# Autodesk Inventor assembly: SPE1V1 Estructura
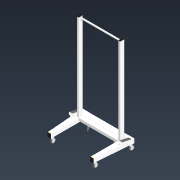
[picture p0: Inventor's stored thumbnail of the model, 180x180]
Saved by Autodesk Inventor 2021.2 (Build 252289000, 289)
## iProperties
Created: 2026-06-02
Part Number: SPE1V1 Estructura
Document SubType Name: Assembly
Designer: nelso
Mass: 32774.5 g
Surface Area: 45303.3 cm^2
Volume: 6303.93 cm^3
Density: 5.19906 g/cm^3
Author: nelso
## Documents named in this file (22)
- C:\Users\Tecnica\OneDrive\Documentos\Mecanica\Soporte-Paciente-Espinografia\Workspace\SPE1V1 Estructura.iam
- C:\Users\Tecnica\OneDrive\Documentos\Mecanica\Soporte-Paciente-Espinografia\Workspace\SP19V1 Tapacanto Delantero.ipt
- C:\Users\Tecnica\OneDrive\Documentos\Mecanica\Soporte-Paciente-Espinografia\Workspace\SP18V1 Tapacanto Superior.ipt
- C:\Users\Tecnica\OneDrive\Documentos\Mecanica\Soporte-Paciente-Espinografia\Workspace\RFPLUS8PO300.ipt
- C:\Users\Tecnica\OneDrive\Documentos\Mecanica\Soporte-Paciente-Espinografia\Workspace\SP17V1 Varilla Pedal.ipt
- C:\Users\Tecnica\OneDrive\Documentos\Mecanica\Soporte-Paciente-Espinografia\Workspace\SP15V1 Pedal Izquierdo.ipt
- C:\Users\Tecnica\OneDrive\Documentos\Mecanica\Soporte-Paciente-Espinografia\Workspace\SPE3V1 Freno.iam
- C:\Users\Tecnica\OneDrive\Documentos\Mecanica\Soporte-Paciente-Espinografia\Workspace\SP14V1 Pedal Derecho.ipt
- C:\Users\Tecnica\OneDrive\Documentos\Mecanica\Soporte-Paciente-Espinografia\Workspace\G3-100-PPP-RU.ipt
- C:\Users\Tecnica\OneDrive\Documentos\Mecanica\Soporte-Paciente-Espinografia\Workspace\DIN 555A10C.ipt
- C:\Users\Tecnica\OneDrive\Documentos\Mecanica\Soporte-Paciente-Espinografia\Workspace\DIN125-A8,4C.ipt
- C:\Users\Tecnica\OneDrive\Documentos\Mecanica\Soporte-Paciente-Espinografia\Workspace\DIN933M8X1.25L20C.ipt
- C:\Users\Tecnica\OneDrive\Documentos\Mecanica\Soporte-Paciente-Espinografia\Workspace\SP11V1 Planchuela Baranda.ipt
- C:\Users\Tecnica\OneDrive\Documentos\Mecanica\Soporte-Paciente-Espinografia\Workspace\SP52V1 Tubo superior.ipt
- C:\Users\Tecnica\OneDrive\Documentos\Mecanica\Soporte-Paciente-Espinografia\Workspace\SP58V1 Seguro Pedales.ipt
- C:\Users\Tecnica\OneDrive\Documentos\Mecanica\Soporte-Paciente-Espinografia\Workspace\ISO7380M6X1L12I.ipt
- C:\Users\Tecnica\OneDrive\Documentos\Mecanica\Soporte-Paciente-Espinografia\Workspace\DIN137-B6.ipt
- C:\Users\Tecnica\OneDrive\Documentos\Mecanica\Soporte-Paciente-Espinografia\Workspace\ISO7380M4X0.8L12I.ipt
- C:\Users\Tecnica\OneDrive\Documentos\Mecanica\Soporte-Paciente-Espinografia\Workspace\DIN137-B4.ipt
- C:\Users\Tecnica\OneDrive\Documentos\Mecanica\Soporte-Paciente-Espinografia\Workspace\DIN555-5M4X0.8I.ipt
- C:\Users\Tecnica\OneDrive\Documentos\Mecanica\Soporte-Paciente-Espinografia\Workspace\SP59V1 Goma Pedalesl.ipt
- C:\Users\Tecnica\OneDrive\Documentos\Mecanica\Soporte-Paciente-Espinografia\Workspace\SPE61V1 Estructura (soldadura).iam
## Components (69 placed, 21 different names)
1. SP18V1 Tapacanto Superior:1
2. SP18V1 Tapacanto Superior:2
3. SP19V1 Tapacanto Delantero:1
4. SP19V1 Tapacanto Delantero:2
5. RFPLUS8PO300:1
6. RFPLUS8PO300:2
7. RFPLUS8PO300:3
8. RFPLUS8PO300:4
9. RFPLUS8PO300:5
10. RFPLUS8PO300:6
11. SP17V1 Varilla Pedal:1 — Mate:117, Mate:118, Mate:119, Mate:120, Mate:121, Mate:128, Mate:129, Mate:130, Mate:132, Mate:133, Mate:134, Mate:258, Mate:261
12. SP14V1 Pedal Derecho:1 — Mate:128, Mate:129, Mate:130, Mate:132, Mate:200, Mate:251, Mate:252, Mate:253, Mate:292, Mate:293, Mate:294, Mate:295, Mate:296
13. SP15V1 Pedal Izquierdo:1 — Mate:120, Mate:121, Flush:132, Mate:248, Mate:249, Mate:250, Mate:286, Mate:287, Mate:297, Mate:298, Mate:299
14. SPE3V1 Freno:1 [sub-assembly] — Flush:103, Mate:117, Mate:118, Mate:119
15. SPE3V1 Freno:2 [sub-assembly] — Flush:103, Mate:133, Mate:134
16. RFPLUS8PO300:17
17. RFPLUS8PO300:18
18. RFPLUS8PO300:19
19. RFPLUS8PO300:20
20. RFPLUS8PO300:21
21. RFPLUS8PO300:22
22. G3-100-PPP-RU:1
23. G3-100-PPP-RU:2
24. G3-100-PPP-RU:3
25. G3-100-PPP-RU:4
26. DIN 555A10C:1
27. DIN 555A10C:2
28. DIN 555A10C:3
29. DIN 555A10C:4
30. DIN125-A8,4C:1 — Mate:214, Mate:215, Mate:219
31. DIN933M8X1.25L20C:1 — Mate:214, Mate:215, Mate:220, Mate:224
32. SP11V1 Planchuela Baranda:1 — Mate:218, Mate:219, Mate:220, Mate:221
33. DIN125-A8,4C:2 — Mate:216, Mate:217, Mate:218
34. DIN933M8X1.25L20C:2 — Mate:216, Mate:217, Mate:221, Mate:223
35. RFPLUS8PO300:23 — Mate:223
36. RFPLUS8PO300:24 — Mate:224
37. DIN125-A8,4C:3
38. DIN933M8X1.25L20C:3
39. SP11V1 Planchuela Baranda:2 — Mate:241
40. DIN125-A8,4C:4
41. DIN933M8X1.25L20C:4
42. RFPLUS8PO300:25
43. RFPLUS8PO300:26
44. SP52V1 Tubo superior:1 — Mate:240, Mate:241
45. SP58V1 Seguro Pedales:1 — Mate:248, Mate:249, Mate:250, Mate:260, Mate:274, Mate:275, Mate:276, Mate:277
46. SP58V1 Seguro Pedales:2 — Mate:251, Mate:252, Mate:253, Mate:259, Mate:270, Mate:271, Mate:272, Mate:273
47. ISO7380M6X1L12I:1 — Mate:254, Mate:255, Mate:258
48. DIN137-B6:1 — Mate:254, Mate:255, Mate:259
49. ISO7380M6X1L12I:2 — Mate:261
50. DIN137-B6:2 — Mate:260
51. ISO7380M4X0.8L12I:1 — Mate:264, Mate:265, Mate:277, Mate:278, Mate:282
52. ISO7380M4X0.8L12I:2 — Mate:262, Mate:263, Mate:276, Mate:279, Mate:284
53. ISO7380M4X0.8L12I:3 — Mate:266, Mate:267, Mate:273, Mate:281, Mate:288
54. ISO7380M4X0.8L12I:4 — Mate:268, Mate:269, Mate:272, Mate:280, Mate:289
55. DIN137-B4:1 — Mate:262, Mate:263, Mate:275
56. DIN137-B4:2 — Mate:264, Mate:265, Mate:274
57. DIN137-B4:3 — Mate:268, Mate:269, Mate:270
58. DIN137-B4:4 — Mate:266, Mate:267, Mate:271
59. DIN137-B4:5 — Mate:279, Mate:285, Mate:287
60. DIN137-B4:6 — Mate:278, Mate:283, Mate:286
61. DIN137-B4:7 — Mate:280, Mate:290, Mate:293
62. DIN137-B4:8 — Mate:281, Mate:291, Mate:292
63. DIN555-5M4X0.8I:1 — Mate:282, Mate:283
64. DIN555-5M4X0.8I:2 — Mate:284, Mate:285
65. DIN555-5M4X0.8I:3 — Mate:289, Mate:290
66. DIN555-5M4X0.8I:4 — Mate:288, Mate:291
67. SP59V1 Goma Pedalesl:1 — Mate:294, Mate:295, Mate:296
68. SP59V1 Goma Pedalesl:2 — Mate:297, Mate:298, Mate:299
69. SPE61V1 Estructura (soldadura):1 [sub-assembly]
## Relationships (168: Mate 134, Flush 33, Angle 1)
- [Mate]: SP18V1 Tapacanto Superior:1 ↔ SPE61V1 Estructura (soldadura):1
- [Flush]: SP18V1 Tapacanto Superior:1 ↔ SPE61V1 Estructura (soldadura):1
- [Mate]: SP18V1 Tapacanto Superior:1 ↔ SPE61V1 Estructura (soldadura):1
- [Flush]: RFPLUS8PO300:2 ↔ SPE61V1 Estructura (soldadura):1
- [Flush]: RFPLUS8PO300:3 ↔ SPE61V1 Estructura (soldadura):1
- [Flush]: RFPLUS8PO300:4 ↔ SPE61V1 Estructura (soldadura):1
- [Flush]: RFPLUS8PO300:5 ↔ SPE61V1 Estructura (soldadura):1
- [Flush]: RFPLUS8PO300:6 ↔ SPE61V1 Estructura (soldadura):1
- [Mate]: RFPLUS8PO300:5 ↔ SPE61V1 Estructura (soldadura):1
- [Mate]: RFPLUS8PO300:6 ↔ SPE61V1 Estructura (soldadura):1
- [Mate]: RFPLUS8PO300:4 ↔ SPE61V1 Estructura (soldadura):1
- [Mate]: RFPLUS8PO300:3 ↔ SPE61V1 Estructura (soldadura):1
- [Mate]: RFPLUS8PO300:2 ↔ SPE61V1 Estructura (soldadura):1
- [Mate]: RFPLUS8PO300:1 ↔ SPE61V1 Estructura (soldadura):1
- [Flush]: RFPLUS8PO300:1 ↔ SPE61V1 Estructura (soldadura):1
- [Mate]: SPE3V1 Freno:1 ↔ SPE61V1 Estructura (soldadura):1
- [Mate]: SPE3V1 Freno:2 ↔ SPE61V1 Estructura (soldadura):1
- Flush:103: SPE3V1 Freno:1 ↔ SPE3V1 Freno:2
- Mate:117: SP17V1 Varilla Pedal:1 ↔ SPE3V1 Freno:1
- Mate:118: SP17V1 Varilla Pedal:1 ↔ SPE3V1 Freno:1
- Mate:119: SP17V1 Varilla Pedal:1 ↔ SPE3V1 Freno:1
- Mate:120: SP17V1 Varilla Pedal:1 ↔ SP15V1 Pedal Izquierdo:1
- Mate:121: SP17V1 Varilla Pedal:1 ↔ SP15V1 Pedal Izquierdo:1
- [Mate]: SPE3V1 Freno:1 ↔ SPE61V1 Estructura (soldadura):1
- [Mate]: SP17V1 Varilla Pedal:1 ↔ SPE61V1 Estructura (soldadura):1
- [Mate] (100 mm): SPE3V1 Freno:2 ↔ SPE61V1 Estructura (soldadura):1
- [Mate] (100 mm): SPE3V1 Freno:1 ↔ SPE61V1 Estructura (soldadura):1
- Mate:128: SP17V1 Varilla Pedal:1 ↔ SP14V1 Pedal Derecho:1
- Mate:129: SP17V1 Varilla Pedal:1 ↔ SP14V1 Pedal Derecho:1
- Mate:130: SP17V1 Varilla Pedal:1 ↔ SP14V1 Pedal Derecho:1
- Mate:132: SP17V1 Varilla Pedal:1 ↔ SP14V1 Pedal Derecho:1
- Mate:133: SP17V1 Varilla Pedal:1 ↔ SPE3V1 Freno:2
- Mate:134: SP17V1 Varilla Pedal:1 ↔ SPE3V1 Freno:2
- [Flush]: SP18V1 Tapacanto Superior:2 ↔ SPE61V1 Estructura (soldadura):1
- [Mate]: SP18V1 Tapacanto Superior:2 ↔ SPE61V1 Estructura (soldadura):1
- [Mate]: G3-100-PPP-RU:4 ↔ SPE61V1 Estructura (soldadura):1
- [Mate]: SP18V1 Tapacanto Superior:2 ↔ SPE61V1 Estructura (soldadura):1
- [Mate]: RFPLUS8PO300:21 ↔ SPE61V1 Estructura (soldadura):1
- [Mate]: RFPLUS8PO300:22 ↔ SPE61V1 Estructura (soldadura):1
- [Mate]: RFPLUS8PO300:20 ↔ SPE61V1 Estructura (soldadura):1
- [Mate]: RFPLUS8PO300:19 ↔ SPE61V1 Estructura (soldadura):1
- [Mate]: RFPLUS8PO300:18 ↔ SPE61V1 Estructura (soldadura):1
- [Mate]: RFPLUS8PO300:17 ↔ SPE61V1 Estructura (soldadura):1
- [Flush]: RFPLUS8PO300:17 ↔ SPE61V1 Estructura (soldadura):1
- [Flush]: RFPLUS8PO300:18 ↔ SPE61V1 Estructura (soldadura):1
- [Flush]: RFPLUS8PO300:19 ↔ SPE61V1 Estructura (soldadura):1
- [Flush]: RFPLUS8PO300:20 ↔ SPE61V1 Estructura (soldadura):1
- [Flush]: RFPLUS8PO300:21 ↔ SPE61V1 Estructura (soldadura):1
- [Flush]: RFPLUS8PO300:22 ↔ SPE61V1 Estructura (soldadura):1
- [Mate]: DIN 555A10C:3 ↔ SPE61V1 Estructura (soldadura):1
- [Mate]: DIN 555A10C:4 ↔ SPE61V1 Estructura (soldadura):1
- [Mate]: DIN 555A10C:2 ↔ SPE61V1 Estructura (soldadura):1
- [Mate]: DIN 555A10C:1 ↔ SPE61V1 Estructura (soldadura):1
- [Mate]: DIN 555A10C:1 ↔ SPE61V1 Estructura (soldadura):1
- [Mate]: DIN 555A10C:2 ↔ SPE61V1 Estructura (soldadura):1
- [Mate]: DIN 555A10C:3 ↔ SPE61V1 Estructura (soldadura):1
- [Mate]: DIN 555A10C:4 ↔ SPE61V1 Estructura (soldadura):1
- [Flush]: SP17V1 Varilla Pedal:1 ↔ SPE61V1 Estructura (soldadura):1
- [Flush] (7.5 mm): SPE61V1 Estructura (soldadura):1
- [Flush] (7.5 mm): SPE61V1 Estructura (soldadura):1
- Flush:132: SP15V1 Pedal Izquierdo:1
- Mate:200: SP14V1 Pedal Derecho:1
- [Mate]: G3-100-PPP-RU:3 ↔ SPE61V1 Estructura (soldadura):1
- [Mate]: G3-100-PPP-RU:3 ↔ SPE61V1 Estructura (soldadura):1
- [Flush]: G3-100-PPP-RU:3 ↔ SPE61V1 Estructura (soldadura):1
- [Mate]: G3-100-PPP-RU:2 ↔ SPE61V1 Estructura (soldadura):1
- [Mate]: G3-100-PPP-RU:2 ↔ SPE61V1 Estructura (soldadura):1
- [Flush]: G3-100-PPP-RU:2 ↔ SPE61V1 Estructura (soldadura):1
- [Mate]: G3-100-PPP-RU:4 ↔ SPE61V1 Estructura (soldadura):1
- [Flush]: G3-100-PPP-RU:4 ↔ SPE61V1 Estructura (soldadura):1
- [Mate]: G3-100-PPP-RU:1 ↔ SPE61V1 Estructura (soldadura):1
- [Flush]: G3-100-PPP-RU:1 ↔ SPE61V1 Estructura (soldadura):1
- [Mate]: G3-100-PPP-RU:1 ↔ SPE61V1 Estructura (soldadura):1
- [Mate]: SP19V1 Tapacanto Delantero:1 ↔ SPE61V1 Estructura (soldadura):1
- [Flush]: SPE61V1 Estructura (soldadura):1
- [Mate]: SPE61V1 Estructura (soldadura):1
- [Flush]: SPE61V1 Estructura (soldadura):1
- [Mate] (380 mm): SPE61V1 Estructura (soldadura):1
- [Flush]: SP19V1 Tapacanto Delantero:2 ↔ SPE61V1 Estructura (soldadura):1
- [Flush]: SP19V1 Tapacanto Delantero:2 ↔ SPE61V1 Estructura (soldadura):1
- [Mate]: SP19V1 Tapacanto Delantero:2 ↔ SPE61V1 Estructura (soldadura):1
- [Flush]: SP19V1 Tapacanto Delantero:1 ↔ SPE61V1 Estructura (soldadura):1
- [Flush]: SP19V1 Tapacanto Delantero:1 ↔ SPE61V1 Estructura (soldadura):1
- Mate:214: DIN125-A8,4C:1 ↔ DIN933M8X1.25L20C:1
- Mate:215: DIN125-A8,4C:1 ↔ DIN933M8X1.25L20C:1
- Mate:216: DIN125-A8,4C:2 ↔ DIN933M8X1.25L20C:2
- Mate:217: DIN125-A8,4C:2 ↔ DIN933M8X1.25L20C:2
- Mate:218: SP11V1 Planchuela Baranda:1 ↔ DIN125-A8,4C:2
- Mate:219: DIN125-A8,4C:1 ↔ SP11V1 Planchuela Baranda:1
- Mate:220: DIN933M8X1.25L20C:1 ↔ SP11V1 Planchuela Baranda:1
- Mate:221: SP11V1 Planchuela Baranda:1 ↔ DIN933M8X1.25L20C:2
- [Mate]: SP11V1 Planchuela Baranda:1 ↔ SPE61V1 Estructura (soldadura):1
- [Flush]: RFPLUS8PO300:24 ↔ SPE61V1 Estructura (soldadura):1
- [Flush]: RFPLUS8PO300:23 ↔ SPE61V1 Estructura (soldadura):1
- Mate:223: DIN933M8X1.25L20C:2 ↔ RFPLUS8PO300:23
- Mate:224: DIN933M8X1.25L20C:1 ↔ RFPLUS8PO300:24
- [Mate]: DIN125-A8,4C:3 ↔ DIN933M8X1.25L20C:3
- [Mate]: DIN125-A8,4C:3 ↔ DIN933M8X1.25L20C:3
- [Mate]: DIN125-A8,4C:4 ↔ DIN933M8X1.25L20C:4
- [Mate]: DIN125-A8,4C:4 ↔ DIN933M8X1.25L20C:4
- [Mate]: SP11V1 Planchuela Baranda:2 ↔ DIN125-A8,4C:4
- [Mate]: DIN125-A8,4C:3 ↔ SP11V1 Planchuela Baranda:2
- [Mate]: DIN933M8X1.25L20C:3 ↔ SP11V1 Planchuela Baranda:2
- [Mate]: SP11V1 Planchuela Baranda:2 ↔ DIN933M8X1.25L20C:4
- [Mate]: DIN933M8X1.25L20C:4 ↔ RFPLUS8PO300:25
- [Mate]: DIN933M8X1.25L20C:3 ↔ RFPLUS8PO300:26
- [Mate]: SP11V1 Planchuela Baranda:2 ↔ SPE61V1 Estructura (soldadura):1
- [Flush]: RFPLUS8PO300:26 ↔ SPE61V1 Estructura (soldadura):1
- [Flush]: RFPLUS8PO300:25 ↔ SPE61V1 Estructura (soldadura):1
- [Mate]: DIN933M8X1.25L20C:1 ↔ SPE61V1 Estructura (soldadura):1
- [Mate]: DIN933M8X1.25L20C:2 ↔ SPE61V1 Estructura (soldadura):1
- [Mate]: DIN933M8X1.25L20C:3 ↔ SPE61V1 Estructura (soldadura):1
- [Mate]: DIN933M8X1.25L20C:4 ↔ SPE61V1 Estructura (soldadura):1
- Mate:240: SP52V1 Tubo superior:1
- Mate:241: SP11V1 Planchuela Baranda:2 ↔ SP52V1 Tubo superior:1
- Mate:248: SP15V1 Pedal Izquierdo:1 ↔ SP58V1 Seguro Pedales:1
- Mate:249: SP15V1 Pedal Izquierdo:1 ↔ SP58V1 Seguro Pedales:1
- Mate:250: SP15V1 Pedal Izquierdo:1 ↔ SP58V1 Seguro Pedales:1
- Mate:251: SP14V1 Pedal Derecho:1 ↔ SP58V1 Seguro Pedales:2
- Mate:252: SP14V1 Pedal Derecho:1 ↔ SP58V1 Seguro Pedales:2
- Mate:253: SP14V1 Pedal Derecho:1 ↔ SP58V1 Seguro Pedales:2
- Mate:254: ISO7380M6X1L12I:1 ↔ DIN137-B6:1
- Mate:255: ISO7380M6X1L12I:1 ↔ DIN137-B6:1
- [Mate]: ISO7380M6X1L12I:2 ↔ DIN137-B6:2
- [Mate]: ISO7380M6X1L12I:2 ↔ DIN137-B6:2
- Mate:258: SP17V1 Varilla Pedal:1 ↔ ISO7380M6X1L12I:1
- Mate:259: SP58V1 Seguro Pedales:2 ↔ DIN137-B6:1
- Mate:260: SP58V1 Seguro Pedales:1 ↔ DIN137-B6:2
- Mate:261: SP17V1 Varilla Pedal:1 ↔ ISO7380M6X1L12I:2
- Mate:262: ISO7380M4X0.8L12I:2 ↔ DIN137-B4:1
- Mate:263: ISO7380M4X0.8L12I:2 ↔ DIN137-B4:1
- Mate:264: ISO7380M4X0.8L12I:1 ↔ DIN137-B4:2
- Mate:265: ISO7380M4X0.8L12I:1 ↔ DIN137-B4:2
- Mate:266: ISO7380M4X0.8L12I:3 ↔ DIN137-B4:4
- Mate:267: ISO7380M4X0.8L12I:3 ↔ DIN137-B4:4
- Mate:268: ISO7380M4X0.8L12I:4 ↔ DIN137-B4:3
- Mate:269: ISO7380M4X0.8L12I:4 ↔ DIN137-B4:3
- Mate:270: SP58V1 Seguro Pedales:2 ↔ DIN137-B4:3
- Mate:271: SP58V1 Seguro Pedales:2 ↔ DIN137-B4:4
- Mate:272: SP58V1 Seguro Pedales:2 ↔ ISO7380M4X0.8L12I:4
- Mate:273: SP58V1 Seguro Pedales:2 ↔ ISO7380M4X0.8L12I:3
- Mate:274: SP58V1 Seguro Pedales:1 ↔ DIN137-B4:2
- Mate:275: SP58V1 Seguro Pedales:1 ↔ DIN137-B4:1
- Mate:276: SP58V1 Seguro Pedales:1 ↔ ISO7380M4X0.8L12I:2
- Mate:277: SP58V1 Seguro Pedales:1 ↔ ISO7380M4X0.8L12I:1
- Mate:278: ISO7380M4X0.8L12I:1 ↔ DIN137-B4:6
- Mate:279: ISO7380M4X0.8L12I:2 ↔ DIN137-B4:5
- Mate:280: ISO7380M4X0.8L12I:4 ↔ DIN137-B4:7
- Mate:281: ISO7380M4X0.8L12I:3 ↔ DIN137-B4:8
- Mate:282: ISO7380M4X0.8L12I:1 ↔ DIN555-5M4X0.8I:1
- Mate:283: DIN137-B4:6 ↔ DIN555-5M4X0.8I:1
- Mate:284: ISO7380M4X0.8L12I:2 ↔ DIN555-5M4X0.8I:2
- Mate:285: DIN137-B4:5 ↔ DIN555-5M4X0.8I:2
- Mate:286: SP15V1 Pedal Izquierdo:1 ↔ DIN137-B4:6
- Mate:287: SP15V1 Pedal Izquierdo:1 ↔ DIN137-B4:5
- Mate:288: ISO7380M4X0.8L12I:3 ↔ DIN555-5M4X0.8I:4
- Mate:289: ISO7380M4X0.8L12I:4 ↔ DIN555-5M4X0.8I:3
- Mate:290: DIN137-B4:7 ↔ DIN555-5M4X0.8I:3
- Mate:291: DIN137-B4:8 ↔ DIN555-5M4X0.8I:4
- Mate:292: SP14V1 Pedal Derecho:1 ↔ DIN137-B4:8
- Mate:293: SP14V1 Pedal Derecho:1 ↔ DIN137-B4:7
- [Angle] (0 deg): SP14V1 Pedal Derecho:1 ↔ SPE61V1 Estructura (soldadura):1
- Mate:294: SP14V1 Pedal Derecho:1 ↔ SP59V1 Goma Pedalesl:1
- Mate:295: SP14V1 Pedal Derecho:1 ↔ SP59V1 Goma Pedalesl:1
- Mate:296: SP14V1 Pedal Derecho:1 ↔ SP59V1 Goma Pedalesl:1
- Mate:297: SP15V1 Pedal Izquierdo:1 ↔ SP59V1 Goma Pedalesl:2
- Mate:298: SP15V1 Pedal Izquierdo:1 ↔ SP59V1 Goma Pedalesl:2
- Mate:299: SP15V1 Pedal Izquierdo:1 ↔ SP59V1 Goma Pedalesl:2
## Named parameters: d314_d103 = 0 mm, d315_d104 = 0 mm, d464_d462 = 0 mm, d465_d463 = 0 mm, d466_d449 = 0 mm, d467_d450 = 0 mm, d468_d451 = 0 mm, d469_d452 = 0 mm, d470_d453 = 0 mm, d471_d454 = 0 mm, d472_d455 = 0 mm, d473_d456 = 0 mm, d500_d498 = 0 mm, d501_d499 = 0 mm
